# Autodesk Inventor assembly: wedgeAssembly01smallerToMatch
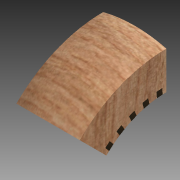
[picture p0: Inventor's stored thumbnail of the model, 180x180]
Saved by Autodesk Inventor 2013 (Build 170138000, 138)
## iProperties
Created: 2013-01-21
Part Number: wedgeAssembly01smallerToMatch
Document SubType Name: Assembly
Designer: Nano
Author: Nano
## Documents named in this file (5)
- C:\Users\Nano\Documents\InventorByron\InventorMasterProject\gyroPhone01\wedgeAssembly01smallerToMatch.iam
- C:\Users\Nano\Documents\InventorByron\InventorMasterProject\gyroPhone01\bigWheelWedge01.ipt
- C:\Users\Nano\Documents\InventorByron\InventorMasterProject\gyroPhone01\magnet1_4x1_4x1_2.ipt
- C:\Users\Nano\Documents\InventorByron\InventorMasterProject\gyroPhone01\magSlotPlugs02.ipt
- C:\Users\Nano\Documents\InventorByron\InventorMasterProject\gyroPhone01\magSlotPlugs03.ipt
## Components (16 placed, 4 different names)
1. bigWheelWedge01:1 — Mate:1, Mate:2, Flush:1, Mate:3, Mate:4, Flush:2, Mate:5, Mate:6, Flush:3
2. magnet1_4x1_4x1_2:1 — Mate:1, Mate:2, Flush:1
3. magnet1_4x1_4x1_2:2
4. magnet1_4x1_4x1_2:3
5. magnet1_4x1_4x1_2:4
6. magnet1_4x1_4x1_2:5
7. magSlotPlugs02:1 — Mate:3, Mate:4, Flush:2
8. magSlotPlugs02:2
9. magSlotPlugs02:3
10. magSlotPlugs02:4
11. magSlotPlugs02:5
12. magSlotPlugs03:1 — Mate:5, Mate:6, Flush:3
13. magSlotPlugs03:2
14. magSlotPlugs03:3
15. magSlotPlugs03:4
16. magSlotPlugs03:5
## Component patterns: (5 elements, first: magnet1_4x1_4x1_2:1), (5 elements, first: magSlotPlugs02:1), (5 elements, first: magSlotPlugs03:1)
## Relationships (9: Mate 6, Flush 3)
- Mate:1: bigWheelWedge01:1 ↔ magnet1_4x1_4x1_2:1
- Mate:2: bigWheelWedge01:1 ↔ magnet1_4x1_4x1_2:1
- Flush:1 (31.75 mm): bigWheelWedge01:1 ↔ magnet1_4x1_4x1_2:1
- Mate:3: bigWheelWedge01:1 ↔ magSlotPlugs02:1
- Mate:4: bigWheelWedge01:1 ↔ magSlotPlugs02:1
- Flush:2: bigWheelWedge01:1 ↔ magSlotPlugs02:1
- Mate:5: bigWheelWedge01:1 ↔ magSlotPlugs03:1
- Mate:6: bigWheelWedge01:1 ↔ magSlotPlugs03:1
- Flush:3: bigWheelWedge01:1 ↔ magSlotPlugs03:1
